# Autodesk Inventor assembly: 2inShooterpipe
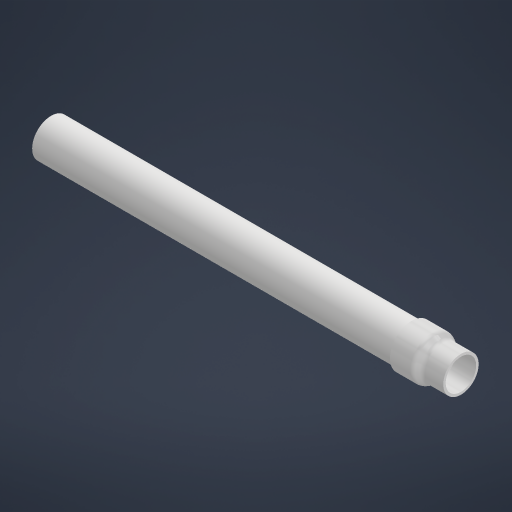
[picture p0: Inventor's stored thumbnail of the model, 512x512]
Saved by Autodesk Inventor 2023 (Build 270158000, 158)
## iProperties
Created: 2022-06-22
Part Number: 2inShooterpipe
Document SubType Name: Assembly
Designer: timmy
Author: timmy
## Documents named in this file (3)
- R:\Inventor\RoboCatz\T-Shirt\Rev2-Better\2inShooterpipe.iam
- R:\Inventor\RoboCatz\T-Shirt\Rev2-Better\2-24inPipw.ipt
- R:\Inventor\RoboCatz\T-Shirt\Rev2-Better\pvc-pipe-fittings-1.snapshot.2\2x1.5in Redicer.ipt
## Components (2 placed, 2 different names)
1. 2-24inPipw:1 — Mate:1, Mate:2
2. 2x1.5in Redicer:1 — Mate:1, Mate:2
## Relationships (2: Mate 2)
- Mate:1: 2-24inPipw:1 ↔ 2x1.5in Redicer:1
- Mate:2: 2-24inPipw:1 ↔ 2x1.5in Redicer:1
